# Autodesk Inventor assembly: MR60 Female
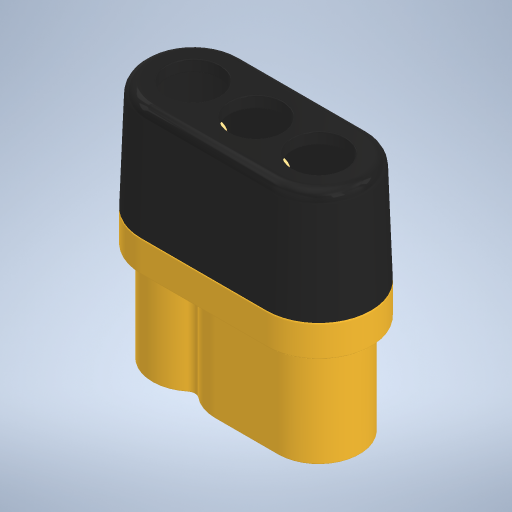
[picture p0: Inventor's stored thumbnail of the model, 512x512]
Saved by Autodesk Inventor 2023 (Build 270158000, 158)
## iProperties
Created: 2021-03-28
Part Number: MR60 Female
Document SubType Name: Assembly
Designer: adamarnold
Sending System: Autodesk Translation Framework v9.10.0.1330
Preprocessor: ST-DEVELOPER v18.1
Title: C:/Users/CG/Downloads/Amass MR60 Female.step
## Documents named in this file (4)
- I:\My Drive\1939\2_Design\2023-2024\Parts\Electronics\Connectors\MR60_Plug.iam
- I:\My Drive\1939\2_Design\2023-2024\Parts\Electronics\Connectors\MR60 Parts\Plug.ipt
- I:\My Drive\1939\2_Design\2023-2024\Parts\Electronics\Connectors\MR60 Parts\Pin.ipt
- I:\My Drive\1939\2_Design\2023-2024\Parts\Electronics\Connectors\MR60 Parts\Cover.ipt
## Components (5 placed, 3 different names)
1. Plug:1 — Mate:2, Mate:3, Mate:4, Flush:1, Angle:1, Angle:2, Angle:3, Mate:5, Mate:6
2. Pin:1 — Flush:2, Flush:3, Angle:2, Mate:6
3. Pin:2 — Mate:1, Mate:2, Flush:1, Angle:1, Flush:2
4. Pin:3 — Flush:3, Angle:3, Mate:5
5. Cover:1 — Mate:1, Mate:3, Mate:4
## Relationships (12: Mate 6, Flush 3, Angle 3)
- Mate:1: Pin:2 ↔ Cover:1
- Mate:2: Plug:1 ↔ Pin:2
- Mate:3: Plug:1 ↔ Cover:1
- Mate:4: Plug:1 ↔ Cover:1
- Flush:1 (-1.4 mm): Plug:1 ↔ Pin:2
- Angle:1 (0 deg): Plug:1 ↔ Pin:2
- Flush:2: Pin:1 ↔ Pin:2
- Flush:3: Pin:1 ↔ Pin:3
- Angle:2 (0 deg): Plug:1 ↔ Pin:1
- Angle:3 (0 deg): Plug:1 ↔ Pin:3
- Mate:5: Plug:1 ↔ Pin:3
- Mate:6: Plug:1 ↔ Pin:1
